# Autodesk Inventor assembly: CH_00_0004_Z128
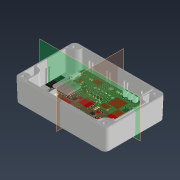
[picture p0: Inventor's stored thumbnail of the model, 180x180]
Saved by Autodesk Inventor 2022.3 (Build 263350030, 350C)
## iProperties
Created: 2022-05-23
Part Number: CH_00_0004_Z128
Document SubType Name: Assembly
Designer: Tomasz Krakowski
Author: Tomasz Krakowski
## iProperties of the stored document Z128.iam
Created: 2018-03-13
Part Number: Z128
Document SubType Name: Assembly
Designer: Tomasz Krakowski
Sending System: Autodesk Inventor 2017
Preprocessor: ST-DEVELOPER v16.5
Title: P:\0.KRADEX\1. Produkty\4. Do wrzucenia na stronę\Z128\Z128_Strona\Z128.stp
Author: przemyslaw.laczynski
## iProperties of the stored document Z128_Base.ipt
Created: 2018-02-09
Part Number: Z128_Base
Material: Generic
Document SubType Name: Modeling
Designer: Tomasz Krakowski
Density: 1 g/cm^3
Appearance: Default
Author: Tomasz Krakowski
Revision Number: ANY
## iProperties of the stored document Z128_Cover.ipt
Created: 2018-02-09
Part Number: Z128_Cover
Material: Generic
Document SubType Name: Modeling
Designer: Tomasz Krakowski
Density: 1 g/cm^3
Appearance: Default
Author: Tomasz Krakowski
Revision Number: ANY
## Documents named in this file (6)
- C:\Repozytoria\sd-roboczy\01_praca\04_model\02_wykonawczy\CH_00_0004_Z128.iam
- **C:\Repozytoria\sd-roboczy\01_praca\04_model\02_wykonawczy\CH_00_0004_Z128.iam*LocalDocs*xAaaaanaaAaaaaaaaAaaaa45mTd*Z128.iam
- C:\Repozytoria\sd-roboczy\01_praca\04_model\02_wykonawczy\CH_01_0051_PCB_layout.ipt
- C:\Repozytoria\sd-roboczy\01_praca\04_model\02_wykonawczy\STEP\Z128.stp
- **C:\Repozytoria\sd-roboczy\01_praca\04_model\02_wykonawczy\CH_00_0004_Z128.iam*LocalDocs*xAaaaa4aaAaaaaaaaAaaaqqdlSg*Z128_Base.ipt
- **C:\Repozytoria\sd-roboczy\01_praca\04_model\02_wykonawczy\CH_00_0004_Z128.iam*LocalDocs*xAaaaaraaAaaaaaaaAaaaqcxh0d*Z128_Cover.ipt
## Components (2 placed, 2 different names)
1. Z128:1 [sub-assembly] — Mate:3
2. CH_01_0051_PCB_layout:1 — Mate:1, Mate:2, Mate:3
## Relationships (3: Mate 3)
- Mate:1: CH_01_0051_PCB_layout:1
- Mate:2 (-1 mm): CH_01_0051_PCB_layout:1
- Mate:3: Z128:1 ↔ CH_01_0051_PCB_layout:1
